# Autodesk Inventor assembly: Gripper Attempt 06
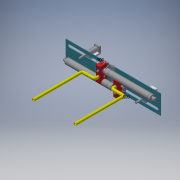
[picture p0: Inventor's stored thumbnail of the model, 180x180]
Saved by Autodesk Inventor 2016 (Build 200138000, 138)
## iProperties
Created: 2015-06-19
Part Number: Gripper Attempt 06
Document SubType Name: Assembly
Designer: steele
Mass: 154531 g
Surface Area: 66016.8 cm^2
Volume: 153238 cm^3
Density: 1.00844 g/cm^3
Author: steele
## Documents named in this file (17)
- C:\snobotics\CAD-Development\robSteele\SnoBoticsSummer2015\Gripper\Gripper Attempt 06.iam
- C:\snobotics\CAD-MfgResources\McMaster-Carr\Air Cylinder\Pivot Mount Cylinders\Foot Bracket for 1_25 and 1_50 Bore\6498K340.ipt
- C:\snobotics\CAD-Development\robSteele\SnoBoticsSummer2015\Gripper\6498K681.ipt
- C:\snobotics\CAD-Development\robSteele\ipartComponents\Plate for Gripper.ipt
- C:\snobotics\CAD-Development\robSteele\SnoBoticsSummer2015\Gripper\Support For Arms.ipt
- C:\snobotics\CAD-Development\robSteele\SnoBoticsSummer2015\Gripper\Support Overlay on Gripper Side.ipt
- C:\snobotics\CAD-Development\robSteele\ipartComponents\ABS Arm.ipt
- C:\snobotics\autodesk\2015\FRC_FieldModel_2015\Parts\YELLOW_TOTE.ipt
- C:\snobotics\autodesk\2015\FRC_FieldModel_2015\Parts\RECYCLING_BIN_ASM.iam
- C:\snobotics\CAD-Development\robSteele\ipartComponents\Plate for Gripper\Plate for Gripper 5.5 x 27 x 1(_FS)8 x 3(_FS)8.ipt
- C:\snobotics\CAD-Development\robSteele\SnoBoticsSummer2015\Gripper\Gripper Attempt 05\Design Accelerator\Bolted Connection1.iam
- C:\snobotics\CAD-Development\robSteele\SnoBoticsSummer2015\Gripper\Gripper Attempt 05\Design Accelerator\Bolted Connection3.iam
- C:\snobotics\CAD-Development\robSteele\SnoBoticsSummer2015\Gripper\Gripper Attempt 05\Design Accelerator\Bolted Connection4.iam
- C:\snobotics\CAD-Development\robSteele\SnoBoticsSummer2015\Gripper\Gripper Attempt 05\Design Accelerator\Bolted Connection5.iam
- C:\snobotics\CAD-Development\robSteele\SnoBoticsSummer2015\Gripper\SupportForStopAirCylinder.ipt
- C:\snobotics\CAD-Development\robSteele\SnoBoticsSummer2015\Gripper\6113K132.ipt
- C:\snobotics\CAD-MfgResources\McMaster-Carr\Air Cylinder\Compact Tie Rod Air Cylinder\Square Face\Stroke 2 in\Bore 1 1_16 in\90985A127.ipt
## Components (24 placed, 12 different names)
1. Plate for Gripper 5.5 x 27 x 1(_FS)8 x 3(_FS)8:1 — Mate:1, Flush:1, Flush:2, Mate:2, Flush:3, Flush:4, Mate:9, Mate:13, Mate:14, Mate:18, Mate:25, Flush:15, Flush:16, Mate:26, Flush:17, Flush:18
2. 6498K340:1 — Mate:2, Flush:3, Flush:4, Mate:7, Mate:17
3. 6498K340:2 — Mate:1, Flush:1, Flush:2, Mate:8
4. 6498K681:1 — Mate:7
5. 6498K681:2 — Mate:8, Insert:3
6. Support For Arms:1 — Mate:9, Insert:3, Mate:10, Flush:10, Flush:13, Mate:12
7. Support For Arms:2 — Mate:13, Mate:14, Mate:15, Flush:14, Mate:16
8. Support Overlay on Gripper Side:1 — Mate:10, Flush:10, Flush:13, Mate:12, Insert:4, Mate:21, Mate:22, Insert:7
9. Support Overlay on Gripper Side:2 — Mate:15, Flush:14, Mate:16, Insert:6, Mate:19, Mate:20, Mate:23, Mate:24, Insert:8
10. ABS Arm:1 — Insert:4
11. ABS Arm:2 — Insert:6
12. 90985A127:1 — Insert:7
13. 90985A127:2 — Insert:8
14. Bolted Connection:1 [sub-assembly] — Mate:17, Mate:18
15. 6113K132:3 — Mate:27, Flush:19, Flush:20
16. 6113K132:4 — Mate:28, Flush:21, Flush:22
17. Bolted Connection:2 [sub-assembly] — Mate:19, Mate:20
18. Bolted Connection:3 [sub-assembly] — Mate:21, Mate:22
19. Bolted Connection:4 [sub-assembly] — Mate:23, Mate:24
20. SupportForStopAirCylinder:1 — Mate:26, Flush:17, Flush:18, Mate:27, Flush:19, Flush:20
21. SupportForStopAirCylinder:2 — Mate:25, Flush:15, Flush:16, Mate:28, Flush:21, Flush:22
22. YELLOW_TOTE:1
23. YELLOW_TOTE:2
24. RECYCLING_BIN_ASM:1 [sub-assembly]
## Relationships (43: Mate 23, Flush 15, Insert 5)
- Mate:1: Plate for Gripper 5.5 x 27 x 1(_FS)8 x 3(_FS)8:1 ↔ 6498K340:2
- Flush:1: Plate for Gripper 5.5 x 27 x 1(_FS)8 x 3(_FS)8:1 ↔ 6498K340:2
- Flush:2 (330.2 mm): Plate for Gripper 5.5 x 27 x 1(_FS)8 x 3(_FS)8:1 ↔ 6498K340:2
- Mate:2: Plate for Gripper 5.5 x 27 x 1(_FS)8 x 3(_FS)8:1 ↔ 6498K340:1
- Flush:3: Plate for Gripper 5.5 x 27 x 1(_FS)8 x 3(_FS)8:1 ↔ 6498K340:1
- Flush:4 (330.2 mm): Plate for Gripper 5.5 x 27 x 1(_FS)8 x 3(_FS)8:1 ↔ 6498K340:1
- Mate:7: 6498K340:1 ↔ 6498K681:1
- Mate:8: 6498K340:2 ↔ 6498K681:2
- Mate:9: Plate for Gripper 5.5 x 27 x 1(_FS)8 x 3(_FS)8:1 ↔ Support For Arms:1
- Insert:3: 6498K681:2 ↔ Support For Arms:1
- Mate:10: Support For Arms:1 ↔ Support Overlay on Gripper Side:1
- Flush:10: Support For Arms:1 ↔ Support Overlay on Gripper Side:1
- Flush:13: Support For Arms:1 ↔ Support Overlay on Gripper Side:1
- Mate:12: Support For Arms:1 ↔ Support Overlay on Gripper Side:1
- Insert:4 (-50.8 mm): Support Overlay on Gripper Side:1 ↔ ABS Arm:1
- Mate:13: Plate for Gripper 5.5 x 27 x 1(_FS)8 x 3(_FS)8:1 ↔ Support For Arms:2
- Mate:14: Plate for Gripper 5.5 x 27 x 1(_FS)8 x 3(_FS)8:1 ↔ Support For Arms:2
- Mate:15: Support For Arms:2 ↔ Support Overlay on Gripper Side:2
- Flush:14: Support For Arms:2 ↔ Support Overlay on Gripper Side:2
- Mate:16: Support For Arms:2 ↔ Support Overlay on Gripper Side:2
- Insert:6 (-50.8 mm): Support Overlay on Gripper Side:2 ↔ ABS Arm:2
- Mate:17: 6498K340:1 ↔ Bolted Connection:1
- Mate:18: Plate for Gripper 5.5 x 27 x 1(_FS)8 x 3(_FS)8:1 ↔ Bolted Connection:1
- Mate:19: Support Overlay on Gripper Side:2 ↔ Bolted Connection:2
- Mate:20: Support Overlay on Gripper Side:2 ↔ Bolted Connection:2
- Mate:21: Support Overlay on Gripper Side:1 ↔ Bolted Connection:3
- Mate:22: Support Overlay on Gripper Side:1 ↔ Bolted Connection:3
- Mate:23: Support Overlay on Gripper Side:2 ↔ Bolted Connection:4
- Mate:24: Support Overlay on Gripper Side:2 ↔ Bolted Connection:4
- Mate:25: Plate for Gripper 5.5 x 27 x 1(_FS)8 x 3(_FS)8:1 ↔ SupportForStopAirCylinder:2
- Flush:15 (-38.1 mm): Plate for Gripper 5.5 x 27 x 1(_FS)8 x 3(_FS)8:1 ↔ SupportForStopAirCylinder:2
- Flush:16 (-120.65 mm): Plate for Gripper 5.5 x 27 x 1(_FS)8 x 3(_FS)8:1 ↔ SupportForStopAirCylinder:2
- Mate:26: Plate for Gripper 5.5 x 27 x 1(_FS)8 x 3(_FS)8:1 ↔ SupportForStopAirCylinder:1
- Flush:17 (-38.1 mm): Plate for Gripper 5.5 x 27 x 1(_FS)8 x 3(_FS)8:1 ↔ SupportForStopAirCylinder:1
- Flush:18 (-120.65 mm): Plate for Gripper 5.5 x 27 x 1(_FS)8 x 3(_FS)8:1 ↔ SupportForStopAirCylinder:1
- Mate:27: 6113K132:3 ↔ SupportForStopAirCylinder:1
- Flush:19: 6113K132:3 ↔ SupportForStopAirCylinder:1
- Flush:20: 6113K132:3 ↔ SupportForStopAirCylinder:1
- Mate:28: 6113K132:4 ↔ SupportForStopAirCylinder:2
- Flush:21: 6113K132:4 ↔ SupportForStopAirCylinder:2
- Flush:22: 6113K132:4 ↔ SupportForStopAirCylinder:2
- Insert:7: Support Overlay on Gripper Side:1 ↔ 90985A127:1
- Insert:8: Support Overlay on Gripper Side:2 ↔ 90985A127:2
## Named parameters: offsetToFrontOfAirCylinder = 330.2 mm, stopDistance = -120.65 mm, distanceForSupport = -38.1 mm
